# Autodesk Inventor assembly: パネル型スカラアームMISUMIアルミフレーム作成Ver
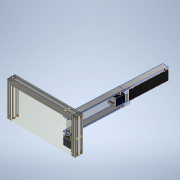
[picture p0: Inventor's stored thumbnail of the model, 180x180]
Saved by Autodesk Inventor 2022 (Build 260153000, 153)
## iProperties
Created: 2022-12-05
Part Number: パネル型スカラアームMISUMIアルミフレーム作成Ver
Document SubType Name: Assembly
Designer: tdn82
Author: tdn82
## Documents named in this file (29)
- C:\Users\tdn82\OneDrive\ドキュメント\Inventor\卒業研究パネル型スカラアーム\GrabCAD\panel-type-scalar-arm\パネル型スカラアーム\パネル型スカラアームMISUMIアルミフレーム作成Ver.iam
- C:\Users\tdn82\OneDrive\ドキュメント\Inventor\卒業研究パネル型スカラアーム\GrabCAD\panel-type-scalar-arm\パネル型スカラアーム\後ろカバー.ipt
- C:\Users\tdn82\OneDrive\ドキュメント\Inventor\卒業研究パネル型スカラアーム\GrabCAD\panel-type-scalar-arm\パネル型スカラアーム\サーボ固定パーツ３Dプリンタ出力実験\サーボモータ固定用１軸目.ipt
- C:\Users\tdn82\OneDrive\ドキュメント\Inventor\卒業研究パネル型スカラアーム\GrabCAD\panel-type-scalar-arm\パネル型スカラアーム\サーボモータB3M-SC-1170-AB3M1100_scale.ipt
- C:\Users\tdn82\OneDrive\ドキュメント\Inventor\卒業研究パネル型スカラアーム\GrabCAD\panel-type-scalar-arm\パネル型スカラアーム\横長2ndフラットバー上 アルミフレーム用.ipt
- C:\Users\tdn82\OneDrive\ドキュメント\Inventor\卒業研究パネル型スカラアーム\GrabCAD\panel-type-scalar-arm\パネル型スカラアーム\前カバー中盤左アーム固定.ipt
- C:\Users\tdn82\OneDrive\ドキュメント\Inventor\卒業研究パネル型スカラアーム\GrabCAD\panel-type-scalar-arm\パネル型スカラアーム\アルミフリーホーン02137_AluminumFreeHornWithBearing_B3M_6000.ipt
- C:\Users\tdn82\OneDrive\ドキュメント\Inventor\卒業研究パネル型スカラアーム\GrabCAD\panel-type-scalar-arm\パネル型スカラアーム\横長3rdフラットバー下.ipt
- C:\Users\tdn82\OneDrive\ドキュメント\Inventor\卒業研究パネル型スカラアーム\GrabCAD\panel-type-scalar-arm\パネル型スカラアーム\横長2ndフラットバー下 アルミフレーム用.ipt
- C:\Users\tdn82\OneDrive\ドキュメント\Inventor\卒業研究パネル型スカラアーム\GrabCAD\panel-type-scalar-arm\パネル型スカラアーム\前カバー中段右.ipt
- C:\Users\tdn82\OneDrive\ドキュメント\Inventor\卒業研究パネル型スカラアーム\GrabCAD\panel-type-scalar-arm\パネル型スカラアーム\前上カバーサーボ隠し.ipt
- C:\Users\tdn82\OneDrive\ドキュメント\Inventor\卒業研究パネル型スカラアーム\GrabCAD\panel-type-scalar-arm\パネル型スカラアーム\前下カバーサーボ隠し.ipt
- C:\Users\tdn82\OneDrive\ドキュメント\Inventor\卒業研究パネル型スカラアーム\GrabCAD\panel-type-scalar-arm\パネル型スカラアーム\三段目アクリル板.ipt
- C:\Users\tdn82\OneDrive\ドキュメント\Inventor\卒業研究パネル型スカラアーム\GrabCAD\panel-type-scalar-arm\パネル型スカラアーム\HFS5-2040-180-Z5-YA10-YB170-Left.ipt
- C:\Users\tdn82\OneDrive\ドキュメント\Inventor\卒業研究パネル型スカラアーム\GrabCAD\panel-type-scalar-arm\パネル型スカラアーム\CBE5-20.ipt
- C:\Users\tdn82\OneDrive\ドキュメント\Inventor\卒業研究パネル型スカラアーム\GrabCAD\panel-type-scalar-arm\パネル型スカラアーム\CSPPN-ST-M3-6_STEP_AP203AP214\CSPPN-STC-M3-6CSPPN-ST-M3-6_203.ipt
- C:\Users\tdn82\OneDrive\ドキュメント\Inventor\卒業研究パネル型スカラアーム\GrabCAD\panel-type-scalar-arm\パネル型スカラアーム\CSPSL-ST3W-M2_6-10_STEP_AP203AP214\サーボホーンとアーム固定するねじCSPSL-ST3W-M2_6-10_203.ipt
- C:\Users\tdn82\OneDrive\ドキュメント\Inventor\卒業研究パネル型スカラアーム\GrabCAD\panel-type-scalar-arm\パネル型スカラアーム\CSPPN-ST-M2_6-18_STEP_AP203AP214\CSPPN-ST-M2_6-18_203.ipt
- C:\Users\tdn82\OneDrive\ドキュメント\Inventor\卒業研究パネル型スカラアーム\GrabCAD\panel-type-scalar-arm\パネル型スカラアーム\CSPPN-ST-M3-6_STEP_AP203AP214\CSPPN-STC-M3-6CSPPN-ST-M3-10_203 - コピー.ipt
- C:\Users\tdn82\OneDrive\ドキュメント\Inventor\卒業研究パネル型スカラアーム\GrabCAD\panel-type-scalar-arm\パネル型スカラアーム\FL674ZZ.ipt
- C:\Users\tdn82\OneDrive\ドキュメント\Inventor\卒業研究パネル型スカラアーム\GrabCAD\panel-type-scalar-arm\パネル型スカラアーム\サーボ固定パーツ３Dプリンタ出力実験\シャフト4.ipt
- C:\Users\tdn82\OneDrive\ドキュメント\Inventor\卒業研究パネル型スカラアーム\GrabCAD\panel-type-scalar-arm\パネル型スカラアーム\サーボ固定パーツ３Dプリンタ出力実験\シャフト4スペーサ.ipt
- C:\Users\tdn82\OneDrive\ドキュメント\Inventor\卒業研究パネル型スカラアーム\GrabCAD\panel-type-scalar-arm\パネル型スカラアーム\HFS5-2040-180-Z5-YA10-YB99-YC170.ipt
- C:\Users\tdn82\OneDrive\ドキュメント\Inventor\卒業研究パネル型スカラアーム\GrabCAD\panel-type-scalar-arm\パネル型スカラアーム\HFS5-2040-320-TPW.ipt
- C:\Users\tdn82\OneDrive\ドキュメント\Inventor\卒業研究パネル型スカラアーム\GrabCAD\panel-type-scalar-arm\パネル型スカラアーム\CBE5-25.ipt
- C:\Users\tdn82\OneDrive\ドキュメント\Inventor\卒業研究パネル型スカラアーム\GrabCAD\panel-type-scalar-arm\パネル型スカラアーム\HFS5-2040-320-TPW-Z5-YA42_5.ipt
- C:\Users\tdn82\OneDrive\ドキュメント\Inventor\卒業研究パネル型スカラアーム\GrabCAD\panel-type-scalar-arm\パネル型スカラアーム\サーボ固定パーツ３Dプリンタ出力実験\シャフト固定用.ipt
- C:\Users\tdn82\OneDrive\ドキュメント\Inventor\卒業研究パネル型スカラアーム\GrabCAD\panel-type-scalar-arm\パネル型スカラアーム\サーボ固定パーツ３Dプリンタ出力実験\サーボモータ固定用２軸目3mm改_new.ipt
- C:\Users\tdn82\OneDrive\ドキュメント\Inventor\卒業研究パネル型スカラアーム\GrabCAD\panel-type-scalar-arm\パネル型スカラアーム\サーボモータB3M1000_scale.ipt
## Components (72 placed, 28 different names)
1. 後ろカバー:1 — フラッシュ:16, メイト:43, フラッシュ:27, 挿入:141, 挿入:142, 挿入:143, 挿入:144, メイト:50
2. サーボモータ固定用１軸目:1 — 挿入:108, 挿入:109, 挿入:135, 挿入:137, 挿入:138, メイト:54, 挿入:147, 挿入:148, フラッシュ:37
3. サーボモータB3M-SC-1170-AB3M1100_scale:1 — 挿入:107, 挿入:108, 挿入:109
4. サーボモータ固定用２軸目3mm改_new:1 — 挿入:18, 挿入:19, 挿入:75, 挿入:77, 挿入:145, 挿入:146, 挿入:149, メイト:55, 挿入:150, 挿入:151
5. 横長2ndフラットバー上 アルミフレーム用:1 — 挿入:67, 挿入:68, 挿入:69, 挿入:70, 挿入:107, 挿入:110, 挿入:111
6. 前カバー中盤左アーム固定:1 — 挿入:110, 挿入:111, 挿入:112, 挿入:113, 挿入:127, 挿入:128, 挿入:129, 挿入:130, 挿入:131, 挿入:132, 挿入:133, 挿入:134, 挿入:145, 挿入:146, 角度:1
7. サーボモータB3M-SC-1170-AB3M1100_scale:2 — 挿入:17, 挿入:18, 挿入:19, メイト:22, 挿入:32
8. アルミフリーホーン02137_AluminumFreeHornWithBearing_B3M_6000:1 — 挿入:17, メイト:27
9. 横長3rdフラットバー下:1 — フラッシュ:2, メイト:22, 挿入:32, 挿入:59, 挿入:60, 挿入:61, 挿入:62, メイト:51, フラッシュ:35
10. 横長3rdフラットバー下:2 — フラッシュ:2, 挿入:63, 挿入:64, 挿入:65, 挿入:66, メイト:27, メイト:52, フラッシュ:36
11. 横長2ndフラットバー下 アルミフレーム用:1 — 挿入:112, 挿入:113, 挿入:115
12. 前カバー中段右:1 — メイト:39, メイト:45, フラッシュ:28
13. 前上カバーサーボ隠し:1 — メイト:33, メイト:34, フラッシュ:32
14. 前下カバーサーボ隠し:1 — フラッシュ:19, メイト:39, メイト:47, フラッシュ:31
15. 三段目アクリル板:1 — 挿入:85, 挿入:86, 挿入:87, 挿入:88, メイト:51, メイト:52, フラッシュ:35, フラッシュ:36, 角度:1
16. HFS5-2040-180-Z5-YA10-YB170-Left:1 — フラッシュ:16, メイト:33, メイト:34, フラッシュ:19, メイト:46, フラッシュ:29, フラッシュ:30, メイト:47, フラッシュ:31
17. CBE5-25:1
18. CBE5-25:2
19. CBE5-25:3
20. CBE5-25:4
21. CBE5-25:5
22. CBE5-25:6
23. CBE5-25:7
24. CBE5-25:8
25. サーボホーンとアーム固定するねじCSPSL-ST3W-M2_6-10_203:1 — 挿入:59
26. サーボホーンとアーム固定するねじCSPSL-ST3W-M2_6-10_203:2 — 挿入:61
27. サーボホーンとアーム固定するねじCSPSL-ST3W-M2_6-10_203:3 — 挿入:62
28. サーボホーンとアーム固定するねじCSPSL-ST3W-M2_6-10_203:4 — 挿入:60
29. サーボホーンとアーム固定するねじCSPSL-ST3W-M2_6-10_203:5 — 挿入:68
30. サーボホーンとアーム固定するねじCSPSL-ST3W-M2_6-10_203:6 — 挿入:67
31. サーボホーンとアーム固定するねじCSPSL-ST3W-M2_6-10_203:7 — 挿入:69
32. サーボホーンとアーム固定するねじCSPSL-ST3W-M2_6-10_203:8 — 挿入:70
33. サーボホーンとアーム固定するねじCSPSL-ST3W-M2_6-10_203:9 — 挿入:63
34. サーボホーンとアーム固定するねじCSPSL-ST3W-M2_6-10_203:10 — 挿入:64
35. サーボホーンとアーム固定するねじCSPSL-ST3W-M2_6-10_203:11 — 挿入:66
36. サーボホーンとアーム固定するねじCSPSL-ST3W-M2_6-10_203:12 — 挿入:65
37. CSPPN-STC-M3-6CSPPN-ST-M3-6_203:2 — 挿入:132
38. CSPPN-STC-M3-6CSPPN-ST-M3-6_203:3 — 挿入:133
39. CSPPN-STC-M3-6CSPPN-ST-M3-6_203:4 — 挿入:131
40. CSPPN-ST-M2_6-18_203:2 — 挿入:77
41. CSPPN-ST-M2_6-18_203:3 — 挿入:149
42. CSPPN-ST-M2_6-18_203:4 — 挿入:75
43. CSPPN-ST-M2_6-18_203:5 — 挿入:137
44. CSPPN-ST-M2_6-18_203:6 — 挿入:138
45. CSPPN-ST-M2_6-18_203:8 — 挿入:135
46. CSPPN-STC-M3-6CSPPN-ST-M3-10_203 - コピー:1 — 挿入:127
47. CSPPN-STC-M3-6CSPPN-ST-M3-10_203 - コピー:2 — 挿入:128
48. CSPPN-STC-M3-6CSPPN-ST-M3-10_203 - コピー:4 — 挿入:85
49. CSPPN-STC-M3-6CSPPN-ST-M3-10_203 - コピー:5 — 挿入:129
50. CSPPN-STC-M3-6CSPPN-ST-M3-10_203 - コピー:6 — 挿入:130
51. CSPPN-STC-M3-6CSPPN-ST-M3-10_203 - コピー:7 — 挿入:86
52. CSPPN-STC-M3-6CSPPN-ST-M3-10_203 - コピー:8 — 挿入:87
53. CSPPN-STC-M3-6CSPPN-ST-M3-10_203 - コピー:10 — 挿入:88
54. CSPPN-STC-M3-6CSPPN-ST-M3-6_203:5 — 挿入:134
55. FL674ZZ:1 — 挿入:114, 円柱状:1, 挿入:117
56. FL674ZZ:2 — 挿入:115, 円柱状:1, 挿入:118
57. シャフト4:1 — 挿入:116
58. シャフト4スペーサ:1 — 挿入:117, 挿入:118
59. HFS5-2040-180-Z5-YA10-YB99-YC170:1 — メイト:44, 挿入:125, 挿入:126, メイト:45, フラッシュ:28, メイト:48, フラッシュ:33, フラッシュ:34, フラッシュ:37
60. HFS5-2040-320-TPW:1 — メイト:43, フラッシュ:27, メイト:44, メイト:46, フラッシュ:29, フラッシュ:30, フラッシュ:32
61. CBE5-20:1 — 挿入:126
62. CBE5-20:2 — 挿入:125
63. HFS5-2040-320-TPW-Z5-YA42_5:1 — メイト:48, フラッシュ:33, フラッシュ:34, メイト:49, 挿入:139, 挿入:140
64. CBE5-20:3 — 挿入:140, メイト:53
65. CBE5-20:4 — 挿入:139
66. CSPPN-STC-M3-6CSPPN-ST-M3-6_203:6 — 挿入:143
67. CSPPN-STC-M3-6CSPPN-ST-M3-6_203:7 — 挿入:141
68. CSPPN-STC-M3-6CSPPN-ST-M3-6_203:8 — 挿入:144
69. CSPPN-STC-M3-6CSPPN-ST-M3-6_203:9 — 挿入:142
70. サーボモータB3M1000_scale:1 — メイト:54, 挿入:147, 挿入:148
71. サーボモータB3M1000_scale:2 — メイト:55, 挿入:150, 挿入:151
72. シャフト固定用:1 — 挿入:114, 挿入:116, メイト:49, メイト:53
## Relationships (106: Insert 68, Mate 20, Flush 16, CylindricalJoint 1, Angle 1)
- 挿入:17 [Insert]: サーボモータB3M-SC-1170-AB3M1100_scale:2 ↔ アルミフリーホーン02137_AluminumFreeHornWithBearing_B3M_6000:1
- 挿入:18 [Insert]: サーボモータ固定用２軸目3mm改_new:1 ↔ サーボモータB3M-SC-1170-AB3M1100_scale:2
- 挿入:19 [Insert]: サーボモータ固定用２軸目3mm改_new:1 ↔ サーボモータB3M-SC-1170-AB3M1100_scale:2
- フラッシュ:2 [Flush]: 横長3rdフラットバー下:1 ↔ 横長3rdフラットバー下:2
- メイト:22 [Mate]: サーボモータB3M-SC-1170-AB3M1100_scale:2 ↔ 横長3rdフラットバー下:1
- 挿入:32 [Insert]: サーボモータB3M-SC-1170-AB3M1100_scale:2 ↔ 横長3rdフラットバー下:1
- 挿入:59 [Insert]: 横長3rdフラットバー下:1 ↔ サーボホーンとアーム固定するねじCSPSL-ST3W-M2_6-10_203:1
- 挿入:60 [Insert]: 横長3rdフラットバー下:1 ↔ サーボホーンとアーム固定するねじCSPSL-ST3W-M2_6-10_203:4
- 挿入:61 [Insert]: 横長3rdフラットバー下:1 ↔ サーボホーンとアーム固定するねじCSPSL-ST3W-M2_6-10_203:2
- 挿入:62 [Insert]: 横長3rdフラットバー下:1 ↔ サーボホーンとアーム固定するねじCSPSL-ST3W-M2_6-10_203:3
- 挿入:63 [Insert]: 横長3rdフラットバー下:2 ↔ サーボホーンとアーム固定するねじCSPSL-ST3W-M2_6-10_203:9
- 挿入:64 [Insert]: 横長3rdフラットバー下:2 ↔ サーボホーンとアーム固定するねじCSPSL-ST3W-M2_6-10_203:10
- 挿入:65 [Insert]: 横長3rdフラットバー下:2 ↔ サーボホーンとアーム固定するねじCSPSL-ST3W-M2_6-10_203:12
- 挿入:66 [Insert]: 横長3rdフラットバー下:2 ↔ サーボホーンとアーム固定するねじCSPSL-ST3W-M2_6-10_203:11
- 挿入:67 [Insert]: 横長2ndフラットバー上 アルミフレーム用:1 ↔ サーボホーンとアーム固定するねじCSPSL-ST3W-M2_6-10_203:6
- 挿入:68 [Insert]: 横長2ndフラットバー上 アルミフレーム用:1 ↔ サーボホーンとアーム固定するねじCSPSL-ST3W-M2_6-10_203:5
- 挿入:69 [Insert]: 横長2ndフラットバー上 アルミフレーム用:1 ↔ サーボホーンとアーム固定するねじCSPSL-ST3W-M2_6-10_203:7
- 挿入:70 [Insert]: 横長2ndフラットバー上 アルミフレーム用:1 ↔ サーボホーンとアーム固定するねじCSPSL-ST3W-M2_6-10_203:8
- 挿入:75 [Insert]: サーボモータ固定用２軸目3mm改_new:1 ↔ CSPPN-ST-M2_6-18_203:4
- 挿入:77 [Insert]: サーボモータ固定用２軸目3mm改_new:1 ↔ CSPPN-ST-M2_6-18_203:2
- 挿入:85 [Insert]: 三段目アクリル板:1 ↔ CSPPN-STC-M3-6CSPPN-ST-M3-10_203 - コピー:4
- 挿入:86 [Insert]: 三段目アクリル板:1 ↔ CSPPN-STC-M3-6CSPPN-ST-M3-10_203 - コピー:7
- 挿入:87 [Insert]: 三段目アクリル板:1 ↔ CSPPN-STC-M3-6CSPPN-ST-M3-10_203 - コピー:8
- 挿入:88 [Insert]: 三段目アクリル板:1 ↔ CSPPN-STC-M3-6CSPPN-ST-M3-10_203 - コピー:10
- メイト:27 [Mate]: アルミフリーホーン02137_AluminumFreeHornWithBearing_B3M_6000:1 ↔ 横長3rdフラットバー下:2
- [Insert]: HFS5-2040-180-Z5-YA10-YB170-Left:1 ↔ CBE5-25:3
- [Insert]: HFS5-2040-180-Z5-YA10-YB170-Left:1 ↔ CBE5-25:4
- [Insert]: HFS5-2040-180-Z5-YA10-YB170-Left:1 ↔ CBE5-25:2
- [Insert]: HFS5-2040-180-Z5-YA10-YB170-Left:1 ↔ CBE5-25:1
- フラッシュ:16 [Flush]: 後ろカバー:1 ↔ HFS5-2040-180-Z5-YA10-YB170-Left:1
- メイト:33 [Mate]: 前上カバーサーボ隠し:1 ↔ HFS5-2040-180-Z5-YA10-YB170-Left:1
- メイト:34 [Mate]: 前上カバーサーボ隠し:1 ↔ HFS5-2040-180-Z5-YA10-YB170-Left:1
- フラッシュ:19 [Flush]: 前下カバーサーボ隠し:1 ↔ HFS5-2040-180-Z5-YA10-YB170-Left:1
- 挿入:107 [Insert]: サーボモータB3M-SC-1170-AB3M1100_scale:1 ↔ 横長2ndフラットバー上 アルミフレーム用:1
- 挿入:108 [Insert]: サーボモータ固定用１軸目:1 ↔ サーボモータB3M-SC-1170-AB3M1100_scale:1
- 挿入:109 [Insert]: サーボモータ固定用１軸目:1 ↔ サーボモータB3M-SC-1170-AB3M1100_scale:1
- 挿入:110 [Insert]: 横長2ndフラットバー上 アルミフレーム用:1 ↔ 前カバー中盤左アーム固定:1
- 挿入:111 [Insert]: 横長2ndフラットバー上 アルミフレーム用:1 ↔ 前カバー中盤左アーム固定:1
- 挿入:112 [Insert]: 前カバー中盤左アーム固定:1 ↔ 横長2ndフラットバー下 アルミフレーム用:1
- 挿入:113 [Insert]: 前カバー中盤左アーム固定:1 ↔ 横長2ndフラットバー下 アルミフレーム用:1
- 挿入:114 [Insert]: FL674ZZ:1 ↔ シャフト固定用:1
- 挿入:115 [Insert]: 横長2ndフラットバー下 アルミフレーム用:1 ↔ FL674ZZ:2
- 円柱状:1 [CylindricalJoint]: FL674ZZ:1 ↔ FL674ZZ:2
- 挿入:116 [Insert]: シャフト4:1 ↔ シャフト固定用:1
- 挿入:117 [Insert]: FL674ZZ:1 ↔ シャフト4スペーサ:1
- 挿入:118 [Insert]: FL674ZZ:2 ↔ シャフト4スペーサ:1
- メイト:39 [Mate]: 前カバー中段右:1 ↔ 前下カバーサーボ隠し:1
- [Flush]: 後ろカバー:1 ↔ HFS5-2040-180-Z5-YA10-YB99-YC170:1
- [Flush]: 後ろカバー:1 ↔ HFS5-2040-180-Z5-YA10-YB99-YC170:1
- [Mate]: 後ろカバー:1 ↔ HFS5-2040-180-Z5-YA10-YB99-YC170:1
- [Mate]: サーボモータ固定用１軸目:1 ↔ HFS5-2040-180-Z5-YA10-YB99-YC170:1
- [Insert]: CBE5-25:6 ↔ HFS5-2040-180-Z5-YA10-YB99-YC170:1
- [Insert]: CBE5-25:5 ↔ HFS5-2040-180-Z5-YA10-YB99-YC170:1
- [Insert]: CBE5-25:8 ↔ HFS5-2040-180-Z5-YA10-YB99-YC170:1
- [Insert]: CBE5-25:7 ↔ HFS5-2040-180-Z5-YA10-YB99-YC170:1
- メイト:43 [Mate]: 後ろカバー:1 ↔ HFS5-2040-320-TPW:1
- フラッシュ:27 [Flush]: 後ろカバー:1 ↔ HFS5-2040-320-TPW:1
- メイト:44 [Mate]: HFS5-2040-180-Z5-YA10-YB99-YC170:1 ↔ HFS5-2040-320-TPW:1
- 挿入:125 [Insert]: HFS5-2040-180-Z5-YA10-YB99-YC170:1 ↔ CBE5-20:2
- 挿入:126 [Insert]: HFS5-2040-180-Z5-YA10-YB99-YC170:1 ↔ CBE5-20:1
- メイト:45 [Mate]: 前カバー中段右:1 ↔ HFS5-2040-180-Z5-YA10-YB99-YC170:1
- フラッシュ:28 [Flush]: 前カバー中段右:1 ↔ HFS5-2040-180-Z5-YA10-YB99-YC170:1
- メイト:46 [Mate]: HFS5-2040-180-Z5-YA10-YB170-Left:1 ↔ HFS5-2040-320-TPW:1
- フラッシュ:29 [Flush]: HFS5-2040-180-Z5-YA10-YB170-Left:1 ↔ HFS5-2040-320-TPW:1
- フラッシュ:30 [Flush]: HFS5-2040-180-Z5-YA10-YB170-Left:1 ↔ HFS5-2040-320-TPW:1
- メイト:47 [Mate]: 前下カバーサーボ隠し:1 ↔ HFS5-2040-180-Z5-YA10-YB170-Left:1
- フラッシュ:31 [Flush]: 前下カバーサーボ隠し:1 ↔ HFS5-2040-180-Z5-YA10-YB170-Left:1
- フラッシュ:32 [Flush]: 前上カバーサーボ隠し:1 ↔ HFS5-2040-320-TPW:1
- メイト:48 [Mate]: HFS5-2040-180-Z5-YA10-YB99-YC170:1 ↔ HFS5-2040-320-TPW-Z5-YA42_5:1
- フラッシュ:33 [Flush]: HFS5-2040-180-Z5-YA10-YB99-YC170:1 ↔ HFS5-2040-320-TPW-Z5-YA42_5:1
- フラッシュ:34 [Flush]: HFS5-2040-180-Z5-YA10-YB99-YC170:1 ↔ HFS5-2040-320-TPW-Z5-YA42_5:1
- 挿入:127 [Insert]: 前カバー中盤左アーム固定:1 ↔ CSPPN-STC-M3-6CSPPN-ST-M3-10_203 - コピー:1
- 挿入:128 [Insert]: 前カバー中盤左アーム固定:1 ↔ CSPPN-STC-M3-6CSPPN-ST-M3-10_203 - コピー:2
- 挿入:129 [Insert]: 前カバー中盤左アーム固定:1 ↔ CSPPN-STC-M3-6CSPPN-ST-M3-10_203 - コピー:5
- 挿入:130 [Insert]: 前カバー中盤左アーム固定:1 ↔ CSPPN-STC-M3-6CSPPN-ST-M3-10_203 - コピー:6
- 挿入:131 [Insert]: 前カバー中盤左アーム固定:1 ↔ CSPPN-STC-M3-6CSPPN-ST-M3-6_203:4
- 挿入:132 [Insert]: 前カバー中盤左アーム固定:1 ↔ CSPPN-STC-M3-6CSPPN-ST-M3-6_203:2
- 挿入:133 [Insert]: 前カバー中盤左アーム固定:1 ↔ CSPPN-STC-M3-6CSPPN-ST-M3-6_203:3
- 挿入:134 [Insert]: 前カバー中盤左アーム固定:1 ↔ CSPPN-STC-M3-6CSPPN-ST-M3-6_203:5
- 挿入:135 [Insert]: サーボモータ固定用１軸目:1 ↔ CSPPN-ST-M2_6-18_203:8
- 挿入:137 [Insert]: サーボモータ固定用１軸目:1 ↔ CSPPN-ST-M2_6-18_203:5
- 挿入:138 [Insert]: サーボモータ固定用１軸目:1 ↔ CSPPN-ST-M2_6-18_203:6
- メイト:49 [Mate]: HFS5-2040-320-TPW-Z5-YA42_5:1 ↔ シャフト固定用:1
- 挿入:139 [Insert]: HFS5-2040-320-TPW-Z5-YA42_5:1 ↔ CBE5-20:4
- 挿入:140 [Insert]: HFS5-2040-320-TPW-Z5-YA42_5:1 ↔ CBE5-20:3
- 挿入:141 [Insert]: 後ろカバー:1 ↔ CSPPN-STC-M3-6CSPPN-ST-M3-6_203:7
- 挿入:142 [Insert]: 後ろカバー:1 ↔ CSPPN-STC-M3-6CSPPN-ST-M3-6_203:9
- 挿入:143 [Insert]: 後ろカバー:1 ↔ CSPPN-STC-M3-6CSPPN-ST-M3-6_203:6
- 挿入:144 [Insert]: 後ろカバー:1 ↔ CSPPN-STC-M3-6CSPPN-ST-M3-6_203:8
- メイト:50 [Mate]: 後ろカバー:1
- 挿入:145 [Insert]: サーボモータ固定用２軸目3mm改_new:1 ↔ 前カバー中盤左アーム固定:1
- 挿入:146 [Insert]: サーボモータ固定用２軸目3mm改_new:1 ↔ 前カバー中盤左アーム固定:1
- メイト:51 [Mate]: 横長3rdフラットバー下:1 ↔ 三段目アクリル板:1
- メイト:52 [Mate]: 横長3rdフラットバー下:2 ↔ 三段目アクリル板:1
- フラッシュ:35 [Flush]: 横長3rdフラットバー下:1 ↔ 三段目アクリル板:1
- フラッシュ:36 [Flush]: 横長3rdフラットバー下:2 ↔ 三段目アクリル板:1
- 角度:1 [Angle] (0 deg): 前カバー中盤左アーム固定:1 ↔ 三段目アクリル板:1
- メイト:53 [Mate]: CBE5-20:3 ↔ シャフト固定用:1
- メイト:54 [Mate]: サーボモータ固定用１軸目:1 ↔ サーボモータB3M1000_scale:1
- 挿入:147 [Insert]: サーボモータ固定用１軸目:1 ↔ サーボモータB3M1000_scale:1
- 挿入:148 [Insert]: サーボモータ固定用１軸目:1 ↔ サーボモータB3M1000_scale:1
- フラッシュ:37 [Flush]: サーボモータ固定用１軸目:1 ↔ HFS5-2040-180-Z5-YA10-YB99-YC170:1
- 挿入:149 [Insert]: サーボモータ固定用２軸目3mm改_new:1 ↔ CSPPN-ST-M2_6-18_203:3
- メイト:55 [Mate]: サーボモータ固定用２軸目3mm改_new:1 ↔ サーボモータB3M1000_scale:2
- 挿入:150 [Insert]: サーボモータ固定用２軸目3mm改_new:1 ↔ サーボモータB3M1000_scale:2
- 挿入:151 [Insert]: サーボモータ固定用２軸目3mm改_new:1 ↔ サーボモータB3M1000_scale:2
